# Autodesk Inventor assembly: KB33-046-003 - Модуль мотора в сборе
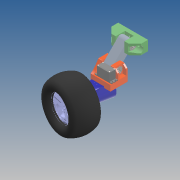
[picture p0: Inventor's stored thumbnail of the model, 180x180]
Saved by Autodesk Inventor 2020 (Build 240168000, 168)
## iProperties
Created: 2021-06-09
Part Number: KB33-046-003 - Модуль мотора в сборе
Material: Типовые
Document SubType Name: Assembly
Designer: Петров Иван
Mass: 1422.86 g
Surface Area: 2186.85 cm^2
Volume: 1363.79 cm^3
Density: 1.04331 g/cm^3
Author: Петров Иван
## Documents named in this file (10)
- E:\IVAN\Ivan_desktop\Kvantorium\Projects\RoboPatrol\design\KB33-046-004 - Динамический модуль мотора в сборе.iam
- E:\IVAN\Ivan_desktop\Kvantorium\Projects\RoboPatrol\design\standart_components\dc_gear_motor_12V_500rpm\dc_gear_motor_12V_500rpm.ipt
- E:\IVAN\Ivan_desktop\Kvantorium\Projects\RoboPatrol\design\KB33-046-004-002 - Крепление к раме.ipt
- E:\IVAN\Ivan_desktop\Kvantorium\Projects\RoboPatrol\design\KB33-046-004-001 - Рычаг.ipt
- E:\IVAN\Ivan_desktop\Kvantorium\Projects\RoboPatrol\design\KB33-046-004-003 - Крепление мотора.ipt
- C:\Users\Петров Иван\Documents\Inventor\Content Center Files\R2020\ru-RU\Bearing 180000 GOST 8882-75\Подшипник 180018 ГОСТ 8882-75.ipt
- E:\IVAN\Ivan_desktop\Kvantorium\Projects\RoboPatrol\design\standart_components\MG996_995\tower prone.ipt
- E:\IVAN\Ivan_desktop\Kvantorium\Projects\RoboPatrol\design\standart_components\WheelBig\колесо большое.iam
- E:\IVAN\Ivan_desktop\Kvantorium\Projects\RoboPatrol\design\KB33-046-004-004 - Крепление мотора.ipt
- E:\IVAN\Ivan_desktop\Kvantorium\Projects\RoboPatrol\design\standart_components\MG996_995\Servo Horn2.ipt
## Components (12 placed, 9 different names)
1. KB33-046-004-002 - Крепление к раме:1 — Совмещение:2, Совмещение:3, Совмещение:7, Совмещение:8, Угол:1, Угол:4
2. KB33-046-004-001 - Рычаг:1 — Совмещение:2, Совмещение:3, Совмещение:4, Совмещение:5, Совмещение:9, Угол:4
3. KB33-046-004-003 - Крепление мотора:1 — Совмещение:4, Совмещение:5, Совмещение:10, Совмещение:11, Совмещение:12, Совмещение:13, Угол:1, Совмещение:19, Совмещение:20, Совмещение:21
4. Подшипник 180000 ГОСТ 8882-75 180018:1 — Совмещение:7
5. Подшипник 180000 ГОСТ 8882-75 180018:2 — Совмещение:8, Совмещение:9
6. Подшипник 180000 ГОСТ 8882-75 180018:3 — Совмещение:10, Совмещение:11
7. Подшипник 180000 ГОСТ 8882-75 180018:4 — Совмещение:12, Совмещение:13
8. dc_gear_motor_12V_500rpm:1 — Совмещение:22, Совмещение:23, Совмещение:24, Совмещение:25, Совмещение:26
9. tower prone:1 — Совмещение:19, Совмещение:20, Совмещение:21, Совмещение:29, Совмещение:30
10. колесо большое:1 [sub-assembly] — Совмещение:22, Совмещение:23
11. KB33-046-004-004 - Крепление мотора:1 — Совмещение:24, Совмещение:25, Совмещение:26, Совмещение:31, Совмещение:32, Совмещение:33
12. Servo Horn2:4 — Совмещение:29, Совмещение:30, Совмещение:31, Совмещение:32, Совмещение:33
## Relationships (26: Mate 24, Angle 2)
- Совмещение:2 [Mate]: KB33-046-004-002 - Крепление к раме:1 ↔ KB33-046-004-001 - Рычаг:1
- Совмещение:3 [Mate]: KB33-046-004-002 - Крепление к раме:1 ↔ KB33-046-004-001 - Рычаг:1
- Совмещение:4 [Mate]: KB33-046-004-001 - Рычаг:1 ↔ KB33-046-004-003 - Крепление мотора:1
- Совмещение:5 [Mate]: KB33-046-004-001 - Рычаг:1 ↔ KB33-046-004-003 - Крепление мотора:1
- Совмещение:7 [Mate]: KB33-046-004-002 - Крепление к раме:1 ↔ Подшипник 180000 ГОСТ 8882-75 180018:1
- Совмещение:8 [Mate]: KB33-046-004-002 - Крепление к раме:1 ↔ Подшипник 180000 ГОСТ 8882-75 180018:2
- Совмещение:9 [Mate]: KB33-046-004-001 - Рычаг:1 ↔ Подшипник 180000 ГОСТ 8882-75 180018:2
- Совмещение:10 [Mate]: KB33-046-004-003 - Крепление мотора:1 ↔ Подшипник 180000 ГОСТ 8882-75 180018:3
- Совмещение:11 [Mate]: KB33-046-004-003 - Крепление мотора:1 ↔ Подшипник 180000 ГОСТ 8882-75 180018:3
- Совмещение:12 [Mate]: KB33-046-004-003 - Крепление мотора:1 ↔ Подшипник 180000 ГОСТ 8882-75 180018:4
- Совмещение:13 [Mate]: KB33-046-004-003 - Крепление мотора:1 ↔ Подшипник 180000 ГОСТ 8882-75 180018:4
- Угол:1 [Angle] (0 deg): KB33-046-004-002 - Крепление к раме:1 ↔ KB33-046-004-003 - Крепление мотора:1
- Угол:4 [Angle] (0 deg): KB33-046-004-002 - Крепление к раме:1 ↔ KB33-046-004-001 - Рычаг:1
- Совмещение:19 [Mate]: KB33-046-004-003 - Крепление мотора:1 ↔ tower prone:1
- Совмещение:20 [Mate]: KB33-046-004-003 - Крепление мотора:1 ↔ tower prone:1
- Совмещение:21 [Mate]: KB33-046-004-003 - Крепление мотора:1 ↔ tower prone:1
- Совмещение:22 [Mate] (40 mm): dc_gear_motor_12V_500rpm:1 ↔ колесо большое:1
- Совмещение:23 [Mate]: dc_gear_motor_12V_500rpm:1 ↔ колесо большое:1
- Совмещение:24 [Mate]: dc_gear_motor_12V_500rpm:1 ↔ KB33-046-004-004 - Крепление мотора:1
- Совмещение:25 [Mate]: dc_gear_motor_12V_500rpm:1 ↔ KB33-046-004-004 - Крепление мотора:1
- Совмещение:26 [Mate]: dc_gear_motor_12V_500rpm:1 ↔ KB33-046-004-004 - Крепление мотора:1
- Совмещение:29 [Mate]: tower prone:1 ↔ Servo Horn2:4
- Совмещение:30 [Mate]: tower prone:1 ↔ Servo Horn2:4
- Совмещение:31 [Mate]: KB33-046-004-004 - Крепление мотора:1 ↔ Servo Horn2:4
- Совмещение:32 [Mate]: KB33-046-004-004 - Крепление мотора:1 ↔ Servo Horn2:4
- Совмещение:33 [Mate]: KB33-046-004-004 - Крепление мотора:1 ↔ Servo Horn2:4
